# Autodesk Inventor assembly: poleAssembly
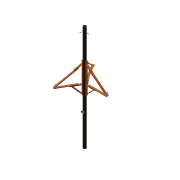
[picture p0: Inventor's stored thumbnail of the model, 180x180]
Saved by Autodesk Inventor 2016 SP2 (Build 200236200, 236)
## iProperties
Created: 2014-08-25
Part Number: poleAssembly
Document SubType Name: Assembly
Designer: Dave
Author: Dave
## Documents named in this file (11)
- C:\Users\krosie\Google Drive\HERA\hera-cad\support\pole\poleAssembly.iam
- C:\Users\krosie\Google Drive\HERA\hera-cad\support\pole\pole.ipt
- C:\Users\krosie\Google Drive\HERA\hera-cad\support\heightMarker.ipt
- C:\Users\krosie\Google Drive\HERA\hera-cad\support\pole\poleStandVertAssy.iam
- C:\Users\krosie\Google Drive\HERA\hera-cad\support\pole\poleStandHorizAssy.iam
- C:\Users\krosie\Google Drive\HERA\hera-cad\smallParts\eyebolt_ss_375.ipt
- C:\Users\krosie\Google Drive\HERA\hera-cad\smallParts\pulley.ipt
- C:\Users\krosie\Google Drive\HERA\hera-cad\support\winchAssembly.iam
- C:\Users\krosie\Google Drive\HERA\hera-cad\smallParts\eyebolt_small.ipt
- C:\Users\krosie\Google Drive\HERA\hera-cad\support\feedCableStay.iam
- C:\Users\krosie\Google Drive\HERA\hera-cad\surface\Connector.ipt
## Components (23 placed, 10 different names)
1. pole:1 — Insert:1, Mate:4, Flush:2, Insert:2, Insert:3, Mate:5
2. heightMarker:1 — Insert:1, Mate:1
3. eyebolt_small:1 — Insert:3
4. feedCableStay:1 [sub-assembly] — Mate:5, Flush:3
5. winchAssembly:1 [sub-assembly]
6. poleStandHorizAssy:1 [sub-assembly] — Mate:2, Flush:1, Mate:3, Mate:6, Angle:1, Mate:8, Angle:2
7. poleStandVertAssy:1 [sub-assembly] — Mate:1, Mate:2, Flush:1, Mate:3, Mate:4, Flush:2, Flush:3, Mate:7, Mate:9
8. Connector:1 — Mate:8, Angle:2, Mate:9
9. Connector:2 — Mate:6, Angle:1, Mate:7
10. pulley:1
11. eyebolt_ss_375:1 — Insert:2
12. poleStandHorizAssy:2 [sub-assembly]
13. poleStandVertAssy:2 [sub-assembly]
14. Connector:3
15. Connector:4
16. pulley:2
17. eyebolt_ss_375:2
18. poleStandHorizAssy:3 [sub-assembly]
19. poleStandVertAssy:3 [sub-assembly]
20. Connector:5
21. Connector:6
22. pulley:3
23. eyebolt_ss_375:3
## Component patterns: (3 elements, first: poleStandHorizAssy:1 + poleStandVertAssy:1 + Connector:1 + Connector:2 + pulley:1 + eyebolt_ss_375:1)
## Relationships (17: Mate 9, Insert 3, Flush 3, Angle 2)
- Insert:1 (-2140 mm): pole:1 ↔ heightMarker:1
- Mate:1 (932 mm): heightMarker:1 ↔ poleStandVertAssy:1
- Mate:2: poleStandHorizAssy:1 ↔ poleStandVertAssy:1
- Flush:1: poleStandHorizAssy:1 ↔ poleStandVertAssy:1
- Mate:3 (162.56 mm): poleStandHorizAssy:1 ↔ poleStandVertAssy:1
- Mate:4: pole:1 ↔ poleStandVertAssy:1
- Flush:2 (44.6 mm): pole:1 ↔ poleStandVertAssy:1
- Insert:2 (-50.8 mm): pole:1 ↔ eyebolt_ss_375:1
- Insert:3 (-7.62 mm): pole:1 ↔ eyebolt_small:1
- Mate:5: pole:1 ↔ feedCableStay:1
- Flush:3 (304.8 mm): feedCableStay:1 ↔ poleStandVertAssy:1
- Mate:6: poleStandHorizAssy:1 ↔ Connector:2
- Angle:1 (0 deg): poleStandHorizAssy:1 ↔ Connector:2
- Mate:7: poleStandVertAssy:1 ↔ Connector:2
- Mate:8: poleStandHorizAssy:1 ↔ Connector:1
- Angle:2 (0 deg): poleStandHorizAssy:1 ↔ Connector:1
- Mate:9: poleStandVertAssy:1 ↔ Connector:1
